# Autodesk Inventor assembly: P-POD
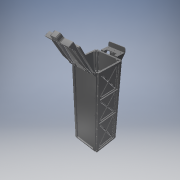
[picture p0: Inventor's stored thumbnail of the model, 180x180]
Saved by Autodesk Inventor 2018 (Build 220112000, 112)
## iProperties
Created: 2018-07-16
Part Number: P-POD
Document SubType Name: Assembly
Designer: Bradley
Author: Bradley
## Documents named in this file (10)
- D:\Users\Bradley\Documents\CougsInSpace\Resources\ComponentModels\Hardware\P-POD.iam
- D:\Users\Bradley\Documents\CougsInSpace\Resources\ComponentModels\Hardware\Components\P-POD\P-POD_Body.ipt
- D:\Users\Bradley\Documents\CougsInSpace\Resources\ComponentModels\Hardware\Components\P-POD\P-POD_Plunger.ipt
- D:\Users\Bradley\Documents\CougsInSpace\Resources\ComponentModels\Hardware\Components\P-POD\P-POD_Spring.ipt
- D:\Users\Bradley\Documents\CougsInSpace\Resources\ComponentModels\Hardware\Components\P-POD\P-POD_Door.ipt
- D:\Users\Bradley\Documents\CougsInSpace\Resources\ComponentModels\Hardware\Components\P-POD\P-POD_DoorSpring.ipt
- D:\Users\Bradley\Documents\CougsInSpace\Resources\ComponentModels\Fasteners\Nut_M4x0.7_3.2mm.ipt
- D:\Users\Bradley\Documents\CougsInSpace\Resources\ComponentModels\Fasteners\Bolt_M4x0.7_35mm_LSH.ipt
- D:\Users\Bradley\Documents\CougsInSpace\Resources\ComponentModels\Hardware\Components\P-POD\P-POD_DoorStop.ipt
- D:\Users\Bradley\Documents\CougsInSpace\Resources\ComponentModels\Fasteners\Bolt_M3x0.35_6mm_LSH.ipt
## Components (53 placed, 9 different names)
1. P-POD_Body:1 — Mate:1, Mate:2, Mate:3, Flush:6, Insert:1, Angle:1, Mate:5, Mate:6, Insert:2, Insert:3, Insert:4, Insert:5, Insert:6, Insert:7, Insert:8, Insert:9, Insert:10, Insert:11
2. P-POD_Plunger:1 — Mate:1, Mate:2, Mate:3, Mate:4
3. P-POD_Spring:1 — Mate:4, Flush:6
4. P-POD_Door:1 — Insert:1, Angle:1, Flush:7, Flush:8
5. P-POD_DoorSpring:1 — Mate:5, Flush:7
6. P-POD_DoorSpring:2 — Mate:6, Flush:8
7. Nut_M4x0.7_3.2mm:1 — Insert:4
8. Nut_M4x0.7_3.2mm:2 — Insert:5
9. Bolt_M4x0.7_35mm_LSH:1 — Insert:3
10. Bolt_M4x0.7_35mm_LSH:2 — Insert:2
11. P-POD_DoorStop:1 — Insert:6, Insert:7, Insert:12, Insert:13
12. Bolt_M3x0.35_6mm_LSH:3 — Insert:13
13. Bolt_M3x0.35_6mm_LSH:6 — Insert:12
14. Bolt_M3x0.35_6mm_LSH:1 — Insert:8
15. Bolt_M3x0.35_6mm_LSH:5 — Insert:11
16. Bolt_M3x0.35_6mm_LSH:2 — Insert:9
17. Bolt_M3x0.35_6mm_LSH:4 — Insert:10
18. Bolt_M3x0.35_6mm_LSH:7
19. Bolt_M3x0.35_6mm_LSH:8
20. Bolt_M3x0.35_6mm_LSH:9
21. Bolt_M3x0.35_6mm_LSH:10
22. Bolt_M3x0.35_6mm_LSH:11
23. Bolt_M3x0.35_6mm_LSH:12
24. Bolt_M3x0.35_6mm_LSH:13
25. Bolt_M3x0.35_6mm_LSH:14
26. Bolt_M3x0.35_6mm_LSH:15
27. Bolt_M3x0.35_6mm_LSH:16
28. Bolt_M3x0.35_6mm_LSH:17
29. Bolt_M3x0.35_6mm_LSH:18
30. Bolt_M3x0.35_6mm_LSH:19
31. Bolt_M3x0.35_6mm_LSH:20
32. Bolt_M3x0.35_6mm_LSH:21
33. Bolt_M3x0.35_6mm_LSH:22
34. Bolt_M3x0.35_6mm_LSH:23
35. Bolt_M3x0.35_6mm_LSH:24
36. Bolt_M3x0.35_6mm_LSH:25
37. Bolt_M3x0.35_6mm_LSH:26
38. Bolt_M3x0.35_6mm_LSH:27
39. Bolt_M3x0.35_6mm_LSH:28
40. Bolt_M3x0.35_6mm_LSH:29
41. Bolt_M3x0.35_6mm_LSH:30
42. Bolt_M3x0.35_6mm_LSH:31
43. Bolt_M3x0.35_6mm_LSH:32
44. Bolt_M3x0.35_6mm_LSH:33
45. Bolt_M3x0.35_6mm_LSH:34
46. Bolt_M3x0.35_6mm_LSH:35
47. Bolt_M3x0.35_6mm_LSH:36
48. Bolt_M3x0.35_6mm_LSH:37
49. Bolt_M3x0.35_6mm_LSH:38
50. Bolt_M3x0.35_6mm_LSH:39
51. Bolt_M3x0.35_6mm_LSH:40
52. Bolt_M3x0.35_6mm_LSH:41
53. Bolt_M3x0.35_6mm_LSH:42
## Component patterns: (10 elements, first: Bolt_M3x0.35_6mm_LSH:1 + Bolt_M3x0.35_6mm_LSH:5 + Bolt_M3x0.35_6mm_LSH:2 + Bolt_M3x0.35_6mm_LSH:4)
## Relationships (23: Insert 13, Mate 6, Flush 3, Angle 1)
- Mate:1: P-POD_Body:1 ↔ P-POD_Plunger:1
- Mate:2: P-POD_Body:1 ↔ P-POD_Plunger:1
- Mate:3: P-POD_Body:1 ↔ P-POD_Plunger:1
- Mate:4: P-POD_Plunger:1 ↔ P-POD_Spring:1
- Flush:6 (-1 mm): P-POD_Body:1 ↔ P-POD_Spring:1
- Insert:1: P-POD_Body:1 ↔ P-POD_Door:1
- Angle:1 (-120 deg): P-POD_Body:1 ↔ P-POD_Door:1
- Mate:5: P-POD_Body:1 ↔ P-POD_DoorSpring:1
- Flush:7 (-0.5 mm): P-POD_Door:1 ↔ P-POD_DoorSpring:1
- Mate:6: P-POD_Body:1 ↔ P-POD_DoorSpring:2
- Flush:8 (-0.5 mm): P-POD_Door:1 ↔ P-POD_DoorSpring:2
- Insert:2: P-POD_Body:1 ↔ Bolt_M4x0.7_35mm_LSH:2
- Insert:3: P-POD_Body:1 ↔ Bolt_M4x0.7_35mm_LSH:1
- Insert:4: P-POD_Body:1 ↔ Nut_M4x0.7_3.2mm:1
- Insert:5: P-POD_Body:1 ↔ Nut_M4x0.7_3.2mm:2
- Insert:6: P-POD_Body:1 ↔ P-POD_DoorStop:1
- Insert:7: P-POD_Body:1 ↔ P-POD_DoorStop:1
- Insert:8: P-POD_Body:1 ↔ Bolt_M3x0.35_6mm_LSH:1
- Insert:9: P-POD_Body:1 ↔ Bolt_M3x0.35_6mm_LSH:2
- Insert:10: P-POD_Body:1 ↔ Bolt_M3x0.35_6mm_LSH:4
- Insert:11: P-POD_Body:1 ↔ Bolt_M3x0.35_6mm_LSH:5
- Insert:12: P-POD_DoorStop:1 ↔ Bolt_M3x0.35_6mm_LSH:6
- Insert:13: P-POD_DoorStop:1 ↔ Bolt_M3x0.35_6mm_LSH:3
